# Autodesk Inventor assembly: Assembly1
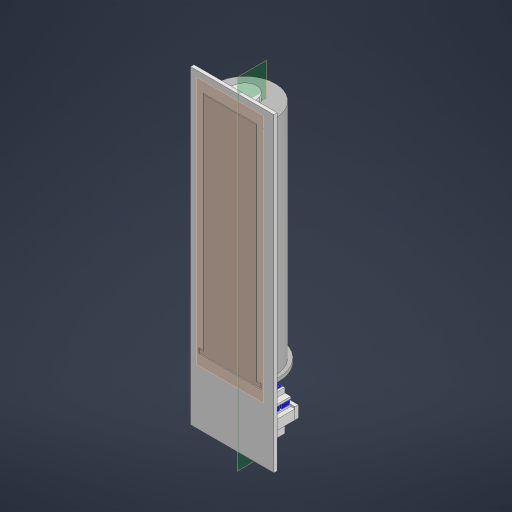
[picture p0: Inventor's stored thumbnail of the model, 512x512]
Saved by Autodesk Inventor 2024.3 (Build 283343000, 343)
## iProperties
Created: 2025-08-14
Part Number: Assembly1
Document SubType Name: Assembly
Designer: giuseppe
Author: giuseppe
## Documents named in this file (5)
- C:\Users\giuseppe\Desktop\Buckshot-Ruolette\CAD\mostra cartucce\Assembly1.iam
- C:\Users\giuseppe\Desktop\Buckshot-Ruolette\CAD\mostra cartucce\rotater shell v3.ipt
- C:\Users\giuseppe\Desktop\Buckshot-Ruolette\CAD\mostra cartucce\SG90 - Micro Servo 9g - Tower Pro.1\SG90 - Micro Servo 9g - Tower Pro.1\SG90 - Micro Servo 9g - Tower Pro.1.ipt
- C:\Users\giuseppe\Desktop\Buckshot-Ruolette\CAD\mostra cartucce\holder.ipt
- C:\Users\giuseppe\Desktop\Buckshot-Ruolette\CAD\mostra cartucce\clip.ipt
## Components (4 placed, 4 different names)
1. rotater shell v3:1 — Mate:1, Mate:2, Flush:1, Flush:2
2. SG90 - Micro Servo 9g - Tower Pro.1:1 — Mate:1, Mate:2
3. holder:1 — Flush:1, Flush:2, Flush:3, Flush:4
4. clip:1 — Flush:3, Flush:4
## Relationships (6: Flush 4, Mate 2)
- Mate:1: rotater shell v3:1 ↔ SG90 - Micro Servo 9g - Tower Pro.1:1
- Mate:2: rotater shell v3:1 ↔ SG90 - Micro Servo 9g - Tower Pro.1:1
- Flush:1: rotater shell v3:1 ↔ holder:1
- Flush:2: rotater shell v3:1 ↔ holder:1
- Flush:3: holder:1 ↔ clip:1
- Flush:4: holder:1 ↔ clip:1
